# Autodesk Inventor assembly: Katownik
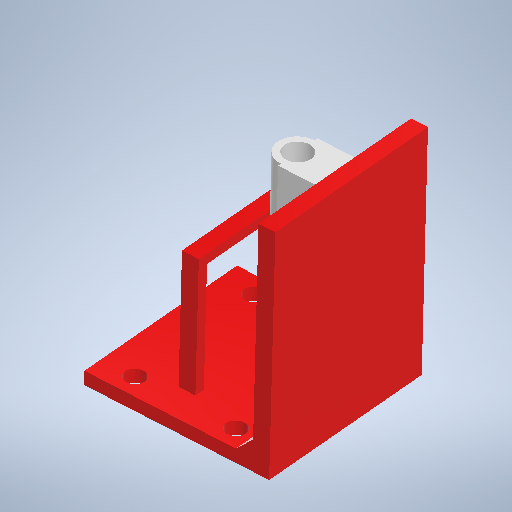
[picture p0: Inventor's stored thumbnail of the model, 512x512]
Saved by Autodesk Inventor 2025 (Build 290162000, 162)
## iProperties
Created: 2024-09-03
Part Number: Katownik
Document SubType Name: Assembly
Designer: user
Author: user
## Documents named in this file (3)
- E:\wazne\kalman-inzynierka\model\Katownik.iam
- E:\wazne\kalman-inzynierka\model\obudowa_łoż_pion_1.ipt
- E:\wazne\kalman-inzynierka\model\chwytak_rurki.ipt
## Components (2 placed, 2 different names)
1. obudowa_łoż_pion_1:1 — Zestawiające:1, Równoległe:1, Równoległe:2
2. chwytak_rurki:1 — Zestawiające:1, Równoległe:1, Równoległe:2
## Relationships (3: Flush 2, Mate 1)
- Zestawiające:1 [Mate]: obudowa_łoż_pion_1:1 ↔ chwytak_rurki:1
- Równoległe:1 [Flush] (20 mm): obudowa_łoż_pion_1:1 ↔ chwytak_rurki:1
- Równoległe:2 [Flush]: obudowa_łoż_pion_1:1 ↔ chwytak_rurki:1
